# Autodesk Inventor assembly: manipulator
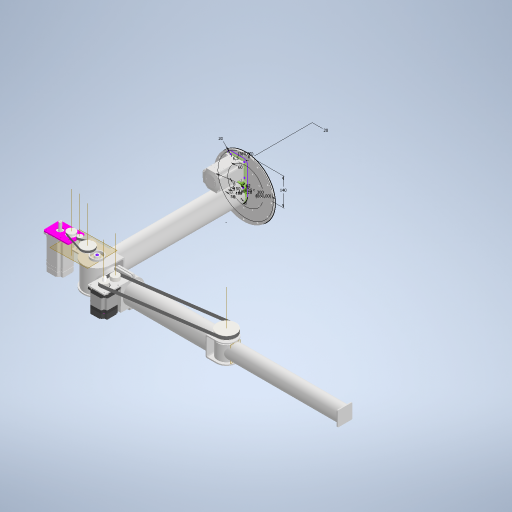
[picture p0: Inventor's stored thumbnail of the model, 512x512]
Saved by Autodesk Inventor 2023 (Build 270158000, 158)
## iProperties
Created: 2023-03-28
Part Number: manipulator
Document SubType Name: Assembly
Designer: krzys
Author: krzys
## Documents named in this file (17)
- C:\Users\krzys\Documents\GitHub\Manipulator-Inventor\Manipulator.iam
- C:\Users\krzys\Documents\GitHub\Manipulator-Inventor\podstawa.ipt
- C:\Users\krzys\Documents\GitHub\Manipulator-Inventor\podstwa_obrotowa.ipt
- C:\Users\krzys\Documents\GitHub\Manipulator-Inventor\CS-M23480_3D.ipt
- C:\Users\krzys\Documents\GitHub\Manipulator-Inventor\czlon 1 i 2.iam
- C:\Users\krzys\Documents\GitHub\Manipulator-Inventor\Manipulator\Design Accelerator\Łożysko6.iam
- C:\Users\krzys\Documents\GitHub\Manipulator-Inventor\Wał2.ipt
- C:\Users\krzys\Documents\GitHub\Manipulator-Inventor\Manipulator\Design Accelerator\Przekładnie walcowe1.iam
- C:\Users\krzys\Documents\GitHub\Manipulator-Inventor\czlon 3.ipt
- C:\Users\krzys\Documents\GitHub\Manipulator-Inventor\mocowanie silnika.ipt
- C:\Users\krzys\Documents\GitHub\Manipulator-Inventor\silniki\CS-M23485B_3D.ipt
- C:\Users\krzys\Documents\GitHub\Manipulator-Inventor\Manipulator\Design Accelerator\Przekładnie pasowe synchroniczne1.iam
- C:\Users\krzys\Documents\GitHub\Manipulator-Inventor\mocowanie_silnika_członu_3.ipt
- C:\Users\krzys\Documents\GitHub\Manipulator-Inventor\Manipulator\Design Accelerator\Przekładnie pasowe synchroniczne2.iam
- C:\Users\krzys\Documents\GitHub\Manipulator-Inventor\silniki\CS-M23445WP\CS-M23445WP_3D.iam
- C:\Users\krzys\Documents\GitHub\Manipulator-Inventor\Manipulator\Design Accelerator\Łożysko5.iam
- C:\Users\krzys\Documents\GitHub\Manipulator-Inventor\podkladka.ipt
## Components (17 placed, 14 different names)
1. podstawa:1 — Wstawiające:6
2. podstwa_obrotowa:1 — Wstawiające:11, Wstawiające:8, Wstawiające:9
3. CS-M23480_3D:1 — Wstawiające:9
4. czlon 1 i 2:1 [sub-assembly] — Wstawiające:11, Wstawiające:1, Zestawiające:6, Wstawiające:2, Równoległe:4, Równoległe:5, Wstawiające:4
5. Łożysko:3 [sub-assembly] — Wstawiające:1, Zestawiające:4, Równoległe:1, Kątowe:1
6. Wał:1 — Zestawiające:4, Równoległe:1, Kątowe:1, Zestawiające:5, Równoległe:2, Równoległe:3
7. Przekładnie walcowe:1 [sub-assembly] — Zestawiające:5, Równoległe:2, Zestawiające:6, Równoległe:3
8. czlon 3:1 — Wstawiające:2
9. mocowanie silnika:1 — Równoległe:4, Równoległe:5, Wstawiające:3
10. CS-M23485B_3D:1 — Wstawiające:3
11. Przekładnie pasowe synchroniczne:1 [sub-assembly]
12. mocowanie_silnika_członu_3:1 — Wstawiające:4, Wstawiające:5
13. Przekładnie pasowe synchroniczne:2 [sub-assembly]
14. CS-M23445WP_3D:1 [sub-assembly] — Wstawiające:5
15. Łożysko:4 [sub-assembly] — Wstawiające:6
16. Łożysko:5 [sub-assembly] — Wstawiające:8, Wstawiające:10
17. podkladka:1 — Wstawiające:10
## Relationships (19: Insert 10, Flush 5, Mate 3, Angle 1)
- Wstawiające:11 [Insert]: podstwa_obrotowa:1 ↔ czlon 1 i 2:1
- Wstawiające:1 [Insert]: czlon 1 i 2:1 ↔ Łożysko:3
- Zestawiające:4 [Mate]: Łożysko:3 ↔ Wał:1
- Równoległe:1 [Flush] (-15 mm): Łożysko:3 ↔ Wał:1
- Kątowe:1 [Angle] (0 deg): Łożysko:3 ↔ Wał:1
- Zestawiające:5 [Mate]: Wał:1 ↔ Przekładnie walcowe:1
- Równoległe:2 [Flush]: Wał:1 ↔ Przekładnie walcowe:1
- Zestawiające:6 [Mate]: czlon 1 i 2:1 ↔ Przekładnie walcowe:1
- Równoległe:3 [Flush]: Wał:1 ↔ Przekładnie walcowe:1
- Wstawiające:2 [Insert] (13.5 mm): czlon 1 i 2:1 ↔ czlon 3:1
- Równoległe:4 [Flush]: czlon 1 i 2:1 ↔ mocowanie silnika:1
- Równoległe:5 [Flush]: czlon 1 i 2:1 ↔ mocowanie silnika:1
- Wstawiające:3 [Insert]: mocowanie silnika:1 ↔ CS-M23485B_3D:1
- Wstawiające:4 [Insert] (-500 mm): czlon 1 i 2:1 ↔ mocowanie_silnika_członu_3:1
- Wstawiające:5 [Insert]: mocowanie_silnika_członu_3:1 ↔ CS-M23445WP_3D:1
- Wstawiające:6 [Insert] (-1 mm): podstawa:1 ↔ Łożysko:4
- Wstawiające:8 [Insert] (1 mm): podstwa_obrotowa:1 ↔ Łożysko:5
- Wstawiające:9 [Insert]: podstwa_obrotowa:1 ↔ CS-M23480_3D:1
- Wstawiające:10 [Insert]: Łożysko:5 ↔ podkladka:1
